# Autodesk Inventor assembly: Return_Spool_Mount
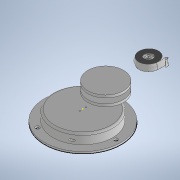
[picture p0: Inventor's stored thumbnail of the model, 180x180]
Saved by Autodesk Inventor 2022 (Build 260153070, 153G)
## iProperties
Created: 2022-03-05
Part Number: Return_Spool_Mount
Document SubType Name: Assembly
Designer: a laptop
Author: a laptop
## Documents named in this file (7)
- C:\Users\a laptop\Desktop\MDL_2021_Project\Return_Spool_Reel\Return_Spool_Mount.iam
- C:\Users\a laptop\Desktop\MDL_2021_Project\Return_Spool_Reel\Return_Spool_Mount.ipt
- C:\Users\a laptop\Desktop\MDL_2021_Project\Return_Spool_Reel\Screws\M8 Washer98689A116_General Purpose 18-8 Stainless Steel Washer.ipt
- C:\Users\a laptop\Desktop\MDL_2021_Project\Return_Spool_Reel\Return_Spool_Mount\Design Accelerator\Bearing2.iam
- C:\Users\a laptop\Desktop\MDL_2021_Project\Return_Spool_Reel\SRM-12-06A.ipt
- C:\Users\a laptop\Desktop\MDL_2021_Project\Return_Spool_Reel\Bearing_Mount.ipt
- C:\Users\a laptop\Desktop\MDL_2021_Project\Return_Spool_Reel\Springs\1842N11_Rotor Spring.ipt
## Components (6 placed, 6 different names)
1. Return_Spool_Mount:1 — Mate:1, Mate:2, Mate:3
2. SRM-12-06A:1 — Mate:1, Mate:2, Mate:3, Mate:4, Mate:5, Mate:6
3. Bearing_Mount:1 — Mate:4, Mate:5, Mate:6, Mate:7, Mate:8, Mate:9
4. Bearing:1 [sub-assembly] — Mate:7, Mate:10
5. M8 Washer98689A116_General Purpose 18-8 Stainless Steel Washer:1 — Mate:8, Mate:9, Mate:10
6. 1842N11_Rotor Spring:1
## Relationships (10: Mate 10)
- Mate:1: Return_Spool_Mount:1 ↔ SRM-12-06A:1
- Mate:2: Return_Spool_Mount:1 ↔ SRM-12-06A:1
- Mate:3: Return_Spool_Mount:1 ↔ SRM-12-06A:1
- Mate:4: SRM-12-06A:1 ↔ Bearing_Mount:1
- Mate:5: SRM-12-06A:1 ↔ Bearing_Mount:1
- Mate:6: SRM-12-06A:1 ↔ Bearing_Mount:1
- Mate:7: Bearing_Mount:1 ↔ Bearing:1
- Mate:8: Bearing_Mount:1 ↔ M8 Washer98689A116_General Purpose 18-8 Stainless Steel Washer:1
- Mate:9: Bearing_Mount:1 ↔ M8 Washer98689A116_General Purpose 18-8 Stainless Steel Washer:1
- Mate:10: Bearing:1 ↔ M8 Washer98689A116_General Purpose 18-8 Stainless Steel Washer:1
